# Autodesk Inventor assembly: Complete7Segment
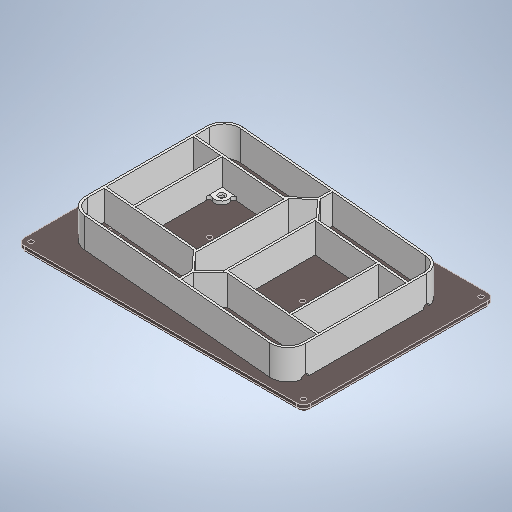
[picture p0: Inventor's stored thumbnail of the model, 512x512]
Saved by Autodesk Inventor 2025.2 (Build 292293000, 293)
## iProperties
Created: 2026-02-06
Part Number: Complete7Segment
Document SubType Name: Assembly
Designer: Joefi
Author: Joefi
## Documents named in this file (4)
- C:\Users\Joefi\Documents\CAD\Inventor\7Segment\Complete7Segment.iam
- C:\Users\Joefi\Documents\CAD\Inventor\7Segment\7Segment.ipt
- C:\Users\Joefi\Documents\CAD\Inventor\7Segment\BackPlate.ipt
- C:\Users\Joefi\Documents\CAD\Inventor\7Segment\Divider.ipt
## Components (3 placed, 3 different names)
1. 7Segment:1 — Mate:1, Mate:2, Flush:1, Flush:2, Mate:4
2. BackPlate:1 — Mate:1, Mate:2, Mate:3, Mate:4
3. Divider:1 — Flush:1, Flush:2, Mate:3
## Relationships (6: Mate 4, Flush 2)
- Mate:1: 7Segment:1 ↔ BackPlate:1
- Mate:2: 7Segment:1 ↔ BackPlate:1
- Flush:1: 7Segment:1 ↔ Divider:1
- Flush:2: 7Segment:1 ↔ Divider:1
- Mate:3: BackPlate:1 ↔ Divider:1
- Mate:4: 7Segment:1 ↔ BackPlate:1
